# Autodesk Inventor assembly: COTS_am-3155 2IN 500Hex Stealth Wheel
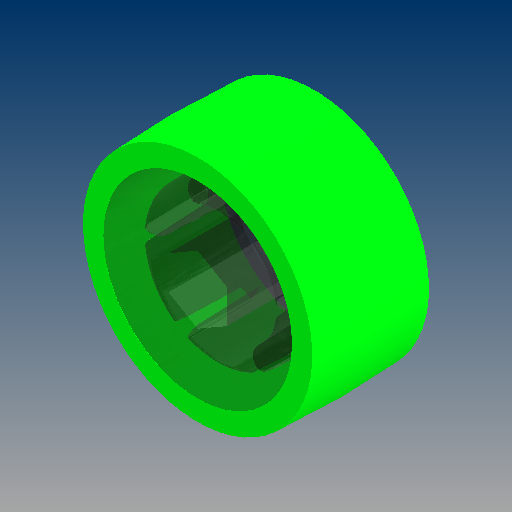
[picture p0: Inventor's stored thumbnail of the model, 512x512]
Saved by Autodesk Inventor 2024.3 (Build 283343000, 343)
## iProperties
Created: 2024-07-30
Part Number: COTS_am-3155 2IN 500Hex Stealth Wheel
Document SubType Name: Assembly
Designer: Bryan
Author: Bryan
## Documents named in this file (3)
- C:\Users\Kenji\Documents\GitHub\1622-2024-Summer-CAD-A-Thon\COTS Library\Motion\Wheels\Stealth Wheels\COTS_am-3155 2IN 500Hex Stealth Wheel.iam
- C:\Users\Kenji\Documents\GitHub\1622-2024-Summer-CAD-A-Thon\COTS Library\Motion\Wheels\Stealth Wheels\COTS_2in Wheel Intergrated 0500 HEX Hub.ipt
- C:\Users\Kenji\Documents\GitHub\1622-2024-Summer-CAD-A-Thon\COTS Library\Motion\Wheels\Stealth Wheels\COTS_2in Tread.ipt
## Components (2 placed, 2 different names)
1. COTS_2in Wheel Intergrated 0500 HEX Hub:1 — Mate:1, Flush:1
2. COTS_2in Tread:1 — Mate:1, Flush:1
## Relationships (2: Mate 1, Flush 1)
- Mate:1: COTS_2in Wheel Intergrated 0500 HEX Hub:1 ↔ COTS_2in Tread:1
- Flush:1: COTS_2in Wheel Intergrated 0500 HEX Hub:1 ↔ COTS_2in Tread:1
